# Autodesk Inventor assembly: nodechimneypanels
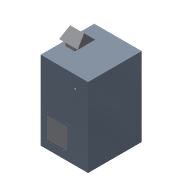
[picture p0: Inventor's stored thumbnail of the model, 180x180]
Saved by Autodesk Inventor 2017 (Build 210142000, 142)
## iProperties
Created: 2016-07-25
Part Number: nodechimneypanels
Document SubType Name: Assembly
Designer: Zuhra Abdurashidova
Author: Zuhra Abdurashidova
## Documents named in this file (7)
- C:\Users\krosie\Google Drive\HERA\hera-cad\Node\nodechimneypanels.iam
- C:\Users\krosie\Google Drive\HERA\hera-cad\Node\EnclosureAssy.iam
- C:\Users\krosie\Google Drive\HERA\hera-cad\Node\plinthScreen.ipt
- C:\Users\krosie\Google Drive\HERA\hera-cad\Node\groundMesh.ipt
- C:\Users\krosie\Google Drive\HERA\hera-cad\Node\chimneyAssy.iam
- C:\Users\krosie\Google Drive\HERA\hera-cad\Node\honeyCombFrame.ipt
- C:\Users\krosie\Google Drive\HERA\hera-cad\Node\8-32ventScrew.ipt
## Components (13 placed, 6 different names)
1. EnclosureAssy:1 [sub-assembly] — Mate:29, Mate:30, Mate:31, Mate:44
2. honeyCombFrame:1
3. plinthBigScreen:1 — Mate:29, Mate:30, Mate:31, Mate:32, Mate:33, Mate:34
4. groundMesh:1 — Mate:32, Mate:33, Mate:34
5. chimneyAssy:1 [sub-assembly] — Mate:44, Mate:49, Mate:50, Angle:1, Mate:51, Angle:2, Mate:52, Mate:53, Mate:54, Mate:55, Mate:56, Mate:57, Mate:59, Mate:60, Mate:61, Mate:62, Mate:63, Angle:3, Angle:4, Angle:5, Angle:6, Angle:7, Mate:64, Mate:65, Angle:8
6. Plain Hex Head Machine Screw - Inch No. 8 - 32 - 1 1/4:1 — Mate:49, Mate:50, Angle:1, Angle:5
7. Plain Hex Head Machine Screw - Inch No. 8 - 32 - 1 1/4:2 — Mate:51, Angle:2, Mate:52
8. Plain Hex Head Machine Screw - Inch No. 8 - 32 - 1 1/4:3 — Mate:56, Mate:60, Angle:6
9. Plain Hex Head Machine Screw - Inch No. 8 - 32 - 1 1/4:4 — Mate:57, Mate:61, Angle:7
10. Plain Hex Head Machine Screw - Inch No. 8 - 32 - 1 1/4:5 — Mate:53, Mate:59
11. Plain Hex Head Machine Screw - Inch No. 8 - 32 - 1 1/4:6 — Mate:54, Mate:62, Angle:3
12. Plain Hex Head Machine Screw - Inch No. 8 - 32 - 1 1/4:7 — Mate:55, Mate:63, Angle:4
13. Plain Hex Head Machine Screw - Inch No. 8 - 32 - 1 1/4:8 — Mate:64, Mate:65, Angle:8
## Relationships (37: Mate 28, Angle 8, Flush 1)
- Mate:29: EnclosureAssy:1 ↔ plinthBigScreen:1
- Mate:30: EnclosureAssy:1 ↔ plinthBigScreen:1
- Mate:31: EnclosureAssy:1 ↔ plinthBigScreen:1
- Mate:32: plinthBigScreen:1 ↔ groundMesh:1
- Mate:33: plinthBigScreen:1 ↔ groundMesh:1
- Mate:34: plinthBigScreen:1 ↔ groundMesh:1
- [Mate]: EnclosureAssy:1 ↔ groundMesh:1
- [Mate]: honeyCombFrame:1 ↔ chimneyAssy:1
- [Mate]: honeyCombFrame:1 ↔ chimneyAssy:1
- Mate:44: EnclosureAssy:1 ↔ chimneyAssy:1
- [Mate]: EnclosureAssy:1 ↔ honeyCombFrame:1
- [Mate]: EnclosureAssy:1 ↔ honeyCombFrame:1
- [Flush]: EnclosureAssy:1 ↔ honeyCombFrame:1
- Mate:49: chimneyAssy:1 ↔ Plain Hex Head Machine Screw - Inch No. 8 - 32 - 1 1/4:1
- Mate:50: chimneyAssy:1 ↔ Plain Hex Head Machine Screw - Inch No. 8 - 32 - 1 1/4:1
- Angle:1 (0 deg): chimneyAssy:1 ↔ Plain Hex Head Machine Screw - Inch No. 8 - 32 - 1 1/4:1
- Mate:51: chimneyAssy:1 ↔ Plain Hex Head Machine Screw - Inch No. 8 - 32 - 1 1/4:2
- Angle:2 (0 deg): chimneyAssy:1 ↔ Plain Hex Head Machine Screw - Inch No. 8 - 32 - 1 1/4:2
- Mate:52: chimneyAssy:1 ↔ Plain Hex Head Machine Screw - Inch No. 8 - 32 - 1 1/4:2
- Mate:53: chimneyAssy:1 ↔ Plain Hex Head Machine Screw - Inch No. 8 - 32 - 1 1/4:5
- Mate:54: chimneyAssy:1 ↔ Plain Hex Head Machine Screw - Inch No. 8 - 32 - 1 1/4:6
- Mate:55: chimneyAssy:1 ↔ Plain Hex Head Machine Screw - Inch No. 8 - 32 - 1 1/4:7
- Mate:56: chimneyAssy:1 ↔ Plain Hex Head Machine Screw - Inch No. 8 - 32 - 1 1/4:3
- Mate:57: chimneyAssy:1 ↔ Plain Hex Head Machine Screw - Inch No. 8 - 32 - 1 1/4:4
- Mate:59: chimneyAssy:1 ↔ Plain Hex Head Machine Screw - Inch No. 8 - 32 - 1 1/4:5
- Mate:60: chimneyAssy:1 ↔ Plain Hex Head Machine Screw - Inch No. 8 - 32 - 1 1/4:3
- Mate:61: chimneyAssy:1 ↔ Plain Hex Head Machine Screw - Inch No. 8 - 32 - 1 1/4:4
- Mate:62: chimneyAssy:1 ↔ Plain Hex Head Machine Screw - Inch No. 8 - 32 - 1 1/4:6
- Mate:63: chimneyAssy:1 ↔ Plain Hex Head Machine Screw - Inch No. 8 - 32 - 1 1/4:7
- Angle:3 (0 deg): chimneyAssy:1 ↔ Plain Hex Head Machine Screw - Inch No. 8 - 32 - 1 1/4:6
- Angle:4 (0 deg): chimneyAssy:1 ↔ Plain Hex Head Machine Screw - Inch No. 8 - 32 - 1 1/4:7
- Angle:5 (0 deg): chimneyAssy:1 ↔ Plain Hex Head Machine Screw - Inch No. 8 - 32 - 1 1/4:1
- Angle:6 (0 deg): chimneyAssy:1 ↔ Plain Hex Head Machine Screw - Inch No. 8 - 32 - 1 1/4:3
- Angle:7 (0 deg): chimneyAssy:1 ↔ Plain Hex Head Machine Screw - Inch No. 8 - 32 - 1 1/4:4
- Mate:64: chimneyAssy:1 ↔ Plain Hex Head Machine Screw - Inch No. 8 - 32 - 1 1/4:8
- Mate:65: chimneyAssy:1 ↔ Plain Hex Head Machine Screw - Inch No. 8 - 32 - 1 1/4:8
- Angle:8 (0 deg): chimneyAssy:1 ↔ Plain Hex Head Machine Screw - Inch No. 8 - 32 - 1 1/4:8
